# Autodesk Inventor assembly: long_link
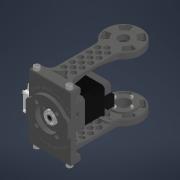
[picture p0: Inventor's stored thumbnail of the model, 180x180]
Saved by Autodesk Inventor 2022 (Build 260153070, 153G)
## iProperties
Created: 2021-11-21
Part Number: long_link
Document SubType Name: Assembly
Designer: Teo
Title: Predstavitev sklopa
Author: Teo
## Documents named in this file (11)
- D:\Zaključna\Roka\Priloge\IPT_files\Assemblies\long_link.iam
- D:\Zaključna\Roka\Priloge\IPT_files\Stepper_nema17.ipt
- D:\Zaključna\Roka\Priloge\IPT_files\Assemblies\reductor_topless.iam
- D:\Zaključna\Roka\Priloge\IPT_files\Stepper_holder_2_lite.ipt
- D:\Zaključna\Roka\Priloge\IPT_files\Forearm_long_1.ipt
- D:\Zaključna\Roka\Priloge\IPT_files\Forearm_long_2.ipt
- D:\Zaključna\Roka\Priloge\IPT_files\Limit_switch.ipt
- C:\Users\Teo\Documents\Inventor\Content Center Files\R2022\en-US\DIN 912\DIN 912 - M2.5 x 0.45 x 4 x 2.875.ipt
- C:\Users\Teo\Documents\Inventor\Content Center Files\R2022\en-US\DIN 912\DIN 912 - M4 x 0.7 x 25 x 23.25.ipt
- C:\Users\Teo\Documents\Inventor\Content Center Files\R2022\en-US\DIN 912\DIN 912 - M5 x 0.8 x 16 x 14.ipt
- C:\Users\Teo\Documents\Inventor\Content Center Files\R2022\en-US\DIN 912\DIN 912 - M4 x 0.7 x 16 x 14.25.ipt
## Components (20 placed, 10 different names)
1. Stepper_nema17:1 — Mate:1, Mate:2, Mate:3
2. reductor_topless:1 [sub-assembly] — Mate:1, Mate:2, Mate:3, Mate:4, Mate:5, Mate:6
3. Stepper_holder_2_lite:1 — Mate:4, Mate:5, Mate:6, Mate:7, Mate:8, Mate:9, Mate:10, Mate:11, Mate:12, Mate:13, Mate:14, Angle:1, Mate:15, Mate:17, Mate:19, Mate:21, Mate:23, Mate:25, Mate:27, Mate:28, Mate:29, Mate:30, Mate:31, Mate:32, Mate:33, Mate:34
4. Forearm_long_1:1 — Mate:7, Mate:8, Mate:9, Mate:20, Mate:22, Mate:35, Mate:36, Mate:37, Mate:38, Mate:39, Mate:40, Mate:41, Mate:42
5. Forearm_long_2:1 — Mate:10, Mate:11, Mate:12, Mate:24, Mate:26
6. Limit_switch:1 — Mate:13, Mate:14, Angle:1, Mate:16, Mate:18
7. DIN 912 - replaced by DIN EN ISO 4762 M2.5 x 4:1 — Mate:15, Mate:16
8. DIN 912 - replaced by DIN EN ISO 4762 M2.5 x 4:2 — Mate:17, Mate:18
9. DIN 912 - replaced by DIN EN ISO 4762 M5 x 16:3 — Mate:19, Mate:20
10. DIN 912 - replaced by DIN EN ISO 4762 M5 x 16:4 — Mate:21, Mate:22
11. DIN 912 - replaced by DIN EN ISO 4762 M5 x 16:2 — Mate:23, Mate:24
12. DIN 912 - replaced by DIN EN ISO 4762 M5 x 16:1 — Mate:25, Mate:26
13. DIN 912 - replaced by DIN EN ISO 4762 M4 x 25:3 — Mate:27, Mate:28
14. DIN 912 - replaced by DIN EN ISO 4762 M4 x 25:4 — Mate:29, Mate:30
15. DIN 912 - replaced by DIN EN ISO 4762 M4 x 25:2 — Mate:31, Mate:32
16. DIN 912 - replaced by DIN EN ISO 4762 M4 x 25:1 — Mate:33, Mate:34
17. DIN 912 - replaced by DIN EN ISO 4762 M4 x 16:2 — Mate:35, Mate:36
18. DIN 912 - replaced by DIN EN ISO 4762 M4 x 16:1 — Mate:37, Mate:38
19. DIN 912 - replaced by DIN EN ISO 4762 M4 x 16:3 — Mate:39, Mate:40
20. DIN 912 - replaced by DIN EN ISO 4762 M4 x 16:4 — Mate:41, Mate:42
## Relationships (43: Mate 42, Angle 1)
- Mate:1: Stepper_nema17:1 ↔ reductor_topless:1
- Mate:2: Stepper_nema17:1 ↔ reductor_topless:1
- Mate:3: Stepper_nema17:1 ↔ reductor_topless:1
- Mate:4: reductor_topless:1 ↔ Stepper_holder_2_lite:1
- Mate:5: reductor_topless:1 ↔ Stepper_holder_2_lite:1
- Mate:6: reductor_topless:1 ↔ Stepper_holder_2_lite:1
- Mate:7: Stepper_holder_2_lite:1 ↔ Forearm_long_1:1
- Mate:8: Stepper_holder_2_lite:1 ↔ Forearm_long_1:1
- Mate:9: Stepper_holder_2_lite:1 ↔ Forearm_long_1:1
- Mate:10: Stepper_holder_2_lite:1 ↔ Forearm_long_2:1
- Mate:11: Stepper_holder_2_lite:1 ↔ Forearm_long_2:1
- Mate:12: Stepper_holder_2_lite:1 ↔ Forearm_long_2:1
- Mate:13: Stepper_holder_2_lite:1 ↔ Limit_switch:1
- Mate:14: Stepper_holder_2_lite:1 ↔ Limit_switch:1
- Angle:1 (0 deg): Stepper_holder_2_lite:1 ↔ Limit_switch:1
- Mate:15: Stepper_holder_2_lite:1 ↔ DIN 912 - replaced by DIN EN ISO 4762 M2.5 x 4:1
- Mate:16: Limit_switch:1 ↔ DIN 912 - replaced by DIN EN ISO 4762 M2.5 x 4:1
- Mate:17: Stepper_holder_2_lite:1 ↔ DIN 912 - replaced by DIN EN ISO 4762 M2.5 x 4:2
- Mate:18: Limit_switch:1 ↔ DIN 912 - replaced by DIN EN ISO 4762 M2.5 x 4:2
- Mate:19: Stepper_holder_2_lite:1 ↔ DIN 912 - replaced by DIN EN ISO 4762 M5 x 16:3
- Mate:20: Forearm_long_1:1 ↔ DIN 912 - replaced by DIN EN ISO 4762 M5 x 16:3
- Mate:21: Stepper_holder_2_lite:1 ↔ DIN 912 - replaced by DIN EN ISO 4762 M5 x 16:4
- Mate:22: Forearm_long_1:1 ↔ DIN 912 - replaced by DIN EN ISO 4762 M5 x 16:4
- Mate:23: Stepper_holder_2_lite:1 ↔ DIN 912 - replaced by DIN EN ISO 4762 M5 x 16:2
- Mate:24: Forearm_long_2:1 ↔ DIN 912 - replaced by DIN EN ISO 4762 M5 x 16:2
- Mate:25: Stepper_holder_2_lite:1 ↔ DIN 912 - replaced by DIN EN ISO 4762 M5 x 16:1
- Mate:26: Forearm_long_2:1 ↔ DIN 912 - replaced by DIN EN ISO 4762 M5 x 16:1
- Mate:27: Stepper_holder_2_lite:1 ↔ DIN 912 - replaced by DIN EN ISO 4762 M4 x 25:3
- Mate:28: Stepper_holder_2_lite:1 ↔ DIN 912 - replaced by DIN EN ISO 4762 M4 x 25:3
- Mate:29: Stepper_holder_2_lite:1 ↔ DIN 912 - replaced by DIN EN ISO 4762 M4 x 25:4
- Mate:30: Stepper_holder_2_lite:1 ↔ DIN 912 - replaced by DIN EN ISO 4762 M4 x 25:4
- Mate:31: Stepper_holder_2_lite:1 ↔ DIN 912 - replaced by DIN EN ISO 4762 M4 x 25:2
- Mate:32: Stepper_holder_2_lite:1 ↔ DIN 912 - replaced by DIN EN ISO 4762 M4 x 25:2
- Mate:33: Stepper_holder_2_lite:1 ↔ DIN 912 - replaced by DIN EN ISO 4762 M4 x 25:1
- Mate:34: Stepper_holder_2_lite:1 ↔ DIN 912 - replaced by DIN EN ISO 4762 M4 x 25:1
- Mate:35: Forearm_long_1:1 ↔ DIN 912 - replaced by DIN EN ISO 4762 M4 x 16:2
- Mate:36: Forearm_long_1:1 ↔ DIN 912 - replaced by DIN EN ISO 4762 M4 x 16:2
- Mate:37: Forearm_long_1:1 ↔ DIN 912 - replaced by DIN EN ISO 4762 M4 x 16:1
- Mate:38: Forearm_long_1:1 ↔ DIN 912 - replaced by DIN EN ISO 4762 M4 x 16:1
- Mate:39: Forearm_long_1:1 ↔ DIN 912 - replaced by DIN EN ISO 4762 M4 x 16:3
- Mate:40: Forearm_long_1:1 ↔ DIN 912 - replaced by DIN EN ISO 4762 M4 x 16:3
- Mate:41: Forearm_long_1:1 ↔ DIN 912 - replaced by DIN EN ISO 4762 M4 x 16:4
- Mate:42: Forearm_long_1:1 ↔ DIN 912 - replaced by DIN EN ISO 4762 M4 x 16:4
